# Autodesk Inventor assembly: Parts to laser cut
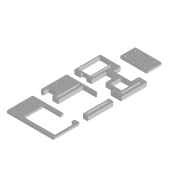
[picture p0: Inventor's stored thumbnail of the model, 180x180]
Saved by Autodesk Inventor 2020 (Build 240168000, 168)
## iProperties
Created: 2021-10-12
Part Number: Parts to laser cut
Document SubType Name: Assembly
Designer: ferrerx
Author: ferrerx
## Documents named in this file (5)
- C:\Users\ferrerx\Documents\GitHub\Sport_Analyzer\Design Files\Mechanical\Parts to laser cut.iam
- C:\Users\ferrerx\Documents\GitHub\Sport_Analyzer\Design Files\Mechanical\Bottom PMMA.ipt
- C:\Users\ferrerx\Documents\GitHub\Sport_Analyzer\Design Files\Mechanical\Middle PMMA.ipt
- C:\Users\ferrerx\Documents\GitHub\Sport_Analyzer\Design Files\Mechanical\Encoder base.ipt
- C:\Users\ferrerx\Documents\GitHub\Sport_Analyzer\Design Files\Mechanical\Top PMMA.ipt
## Components (4 placed, 4 different names)
1. Bottom PMMA:1 — Mate:2, Angle:1
2. Middle PMMA:1 — Mate:3
3. Encoder base:1 — Mate:4, Angle:1
4. Top PMMA:1 — Mate:1
## Relationships (5: Mate 4, Angle 1)
- Mate:1: Top PMMA:1
- Mate:2: Bottom PMMA:1
- Mate:3: Middle PMMA:1
- Mate:4: Encoder base:1
- Angle:1 (0 deg): Bottom PMMA:1 ↔ Encoder base:1
